# Autodesk Inventor assembly: Embeddeck
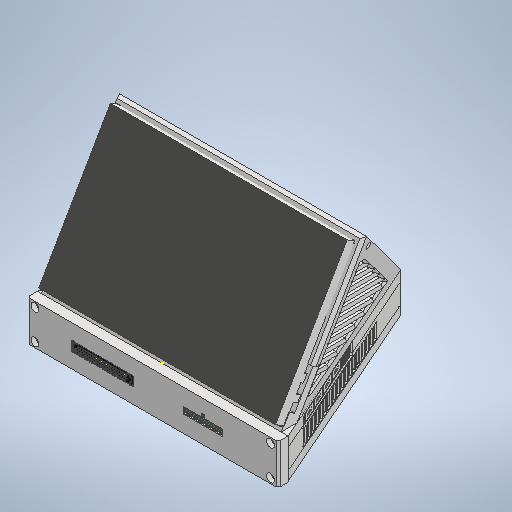
[picture p0: Inventor's stored thumbnail of the model, 512x512]
Saved by Autodesk Inventor 2025.2 (Build 292293000, 293)
## iProperties
Created: 2025-08-07
Part Number: Embeddeck
Document SubType Name: Assembly
Designer: hofma
Author: hofma
## Documents named in this file (14)
- C:\Git\Embeddeck\cad\Embeddeck.iam
- C:\Git\Embeddeck\cad\parts\Digilent Analog Discovery 2\Digilent Analog Discovery 2.iam
- C:\Git\Embeddeck\cad\parts\Raspberry Pi 5\RASPBERRY_PI_5_1.iam
- C:\Git\Embeddeck\cad\parts\Monitor.ipt
- C:\Git\Embeddeck\cad\parts\Conector RIBBON 40 Pins.ipt
- C:\Git\Embeddeck\cad\FrontPlate.ipt
- C:\Git\Embeddeck\cad\parts\PowerUSB.ipt
- C:\Git\Embeddeck\cad\parts\USBextender.ipt
- C:\Git\Embeddeck\cad\BottomPlate.ipt
- C:\Git\Embeddeck\cad\TopPlate.ipt
- C:\Git\Embeddeck\cad\Case.ipt
- C:\Git\Embeddeck\cad\PanelRight.ipt
- C:\Git\Embeddeck\cad\PanelLeft.ipt
- C:\Git\Embeddeck\cad\parts\Fan.ipt
## Components (13 placed, 13 different names)
1. Digilent Analog Discovery 2:1 [sub-assembly] — Mate:5, Flush:5, Flush:6
2. RASPBERRY_PI_5_1:1 [sub-assembly] — Mate:37, Mate:38, Mate:39
3. Monitor:1 — Mate:37, Mate:38, Mate:39, Mate:40
4. Conector RIBBON 40 Pins:1 — Mate:4, Flush:4, Mate:6
5. FrontPlate:1 — Flush:1, Flush:2, Flush:3, Mate:4, Flush:4, Mate:5, Flush:5, Flush:6, Mate:6, Mate:7, Flush:7, Mate:8, Mate:9, Flush:8, Mate:10
6. PowerUSB:1 — Mate:35, Mate:36, Flush:9
7. USBextender:1
8. BottomPlate:1 — Mate:7, Flush:7, Mate:8, Mate:29, Mate:30, Mate:31, Mate:32, Mate:33
9. TopPlate:1 — Mate:9, Flush:8, Mate:10, Mate:18, Mate:19, Mate:34, Mate:35, Flush:9
10. Case:1 — Mate:18, Mate:19, Mate:26, Mate:27, Mate:28, Mate:40
11. PanelRight:1 — Mate:29, Mate:30, Mate:31, Mate:36
12. PanelLeft:1 — Mate:32, Mate:33, Mate:34
13. Fan:1 — Mate:26, Mate:27, Mate:28
## Relationships (33: Mate 24, Flush 9)
- Flush:1: FrontPlate:1
- Flush:2: FrontPlate:1
- Flush:3: FrontPlate:1
- Mate:4: Conector RIBBON 40 Pins:1 ↔ FrontPlate:1
- Flush:4: Conector RIBBON 40 Pins:1 ↔ FrontPlate:1
- Mate:5 (1.35 mm): Digilent Analog Discovery 2:1 ↔ FrontPlate:1
- Flush:5 (2 mm): Digilent Analog Discovery 2:1 ↔ FrontPlate:1
- Flush:6 (-0.335 mm): Digilent Analog Discovery 2:1 ↔ FrontPlate:1
- Mate:6 (0.1 mm): Conector RIBBON 40 Pins:1 ↔ FrontPlate:1
- Mate:7: FrontPlate:1 ↔ BottomPlate:1
- Flush:7: FrontPlate:1 ↔ BottomPlate:1
- Mate:8: FrontPlate:1 ↔ BottomPlate:1
- Mate:9: FrontPlate:1 ↔ TopPlate:1
- Flush:8: FrontPlate:1 ↔ TopPlate:1
- Mate:10: FrontPlate:1 ↔ TopPlate:1
- Mate:18: TopPlate:1 ↔ Case:1
- Mate:19: TopPlate:1 ↔ Case:1
- Mate:26: Case:1 ↔ Fan:1
- Mate:27: Case:1 ↔ Fan:1
- Mate:28: Case:1 ↔ Fan:1
- Mate:29: BottomPlate:1 ↔ PanelRight:1
- Mate:30: BottomPlate:1 ↔ PanelRight:1
- Mate:31: BottomPlate:1 ↔ PanelRight:1
- Mate:32: BottomPlate:1 ↔ PanelLeft:1
- Mate:33: BottomPlate:1 ↔ PanelLeft:1
- Mate:34: TopPlate:1 ↔ PanelLeft:1
- Mate:35: PowerUSB:1 ↔ TopPlate:1
- Mate:36: PowerUSB:1 ↔ PanelRight:1
- Flush:9: PowerUSB:1 ↔ TopPlate:1
- Mate:37: RASPBERRY_PI_5_1:1 ↔ Monitor:1
- Mate:38: RASPBERRY_PI_5_1:1 ↔ Monitor:1
- Mate:39: RASPBERRY_PI_5_1:1 ↔ Monitor:1
- Mate:40: Monitor:1 ↔ Case:1
